# Autodesk Inventor assembly: Bed Leveling Screw
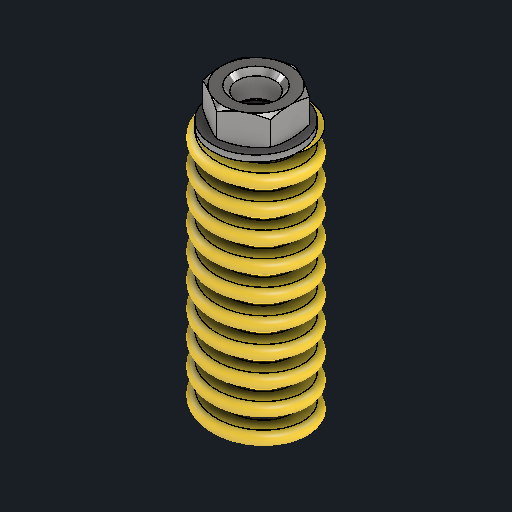
[picture p0: Inventor's stored thumbnail of the model, 512x512]
Saved by Autodesk Inventor 2026.1 (Build 301233020, 233B)
## iProperties
Created: 2025-05-11
Part Number: Bed Leveling Screw
Document SubType Name: Assembly
Designer: Joshua Eah
Author: Joshua Eah
## Documents named in this file (4)
- C:\Users\JoshuaEah\Documents\GitHub\Voron-0\CAD\Z Axis\Subassemblies\Bed Leveling Screw.iam
- C:\Users\JoshuaEah\Documents\GitHub\Voron-0\CAD\Hardware\M3 Hexnut.ipt
- C:\Users\JoshuaEah\Documents\GitHub\Voron-0\CAD\Hardware\M3_Washer.ipt
- C:\Users\JoshuaEah\Documents\GitHub\Voron-0\CAD\Z Axis\Parts\Yellow Die Spring.ipt
## Components (3 placed, 3 different names)
1. M3 Hexnut:1 — Insert:1
2. M3_Washer:1 — Insert:1, Mate:1, Mate:2
3. Yellow Die Spring:1 — Mate:1, Mate:2
## Relationships (3: Mate 2, Insert 1)
- Insert:1: M3 Hexnut:1 ↔ M3_Washer:1
- Mate:1: M3_Washer:1 ↔ Yellow Die Spring:1
- Mate:2: M3_Washer:1 ↔ Yellow Die Spring:1
